# Autodesk Inventor assembly: 42146-11
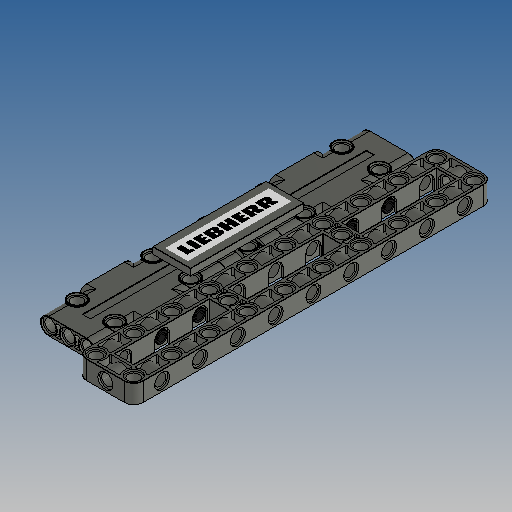
[picture p0: Inventor's stored thumbnail of the model, 512x512]
Saved by Autodesk Inventor 2025 (Build 290162010, 162A)
## iProperties
Created: 2024-11-18
Part Number: 42146-11
Material: Generisch
Document SubType Name: Assembly
Designer: hp.muther
Author: hp.muther
## Documents named in this file (7)
- D:\Inventor\Projekte\Muther\LEGO Technic\LEGO Technik - Raupenkran LR 13000 (42146)\42146-11.iam
- D:\Inventor\Projekte\Muther\LEGO Technic\LEGO Pieces\Verbindungselemente\39793-DkBluishGray.ipt
- D:\Inventor\Projekte\Muther\LEGO Technic\LEGO Pieces\Paneelen\71709-DkBluishGray.ipt
- D:\Inventor\Projekte\Muther\LEGO Technic\LEGO Pieces\Pin's\2780-Black.ipt
- D:\Inventor\Projekte\Muther\LEGO Technic\LEGO Pieces\Pin's\4274-Red.ipt
- D:\Inventor\Projekte\Muther\LEGO Technic\LEGO Pieces\Rahmen, T-Stücke\67491-DkBluishGray.ipt
- D:\Inventor\Projekte\Muther\LEGO Technic\LEGO Technik - Raupenkran LR 13000 (42146)\42146_69729_1.ipt
## Components (15 placed, 6 different names)
1. 39793-DkBluishGray:1 — Einfügen:1, Einfügen:2, Einfügen:3, Einfügen:4, Einfügen:5, Einfügen:6, Einfügen:7, Einfügen:12
2. 71709-DkBluishGray:1 — Einfügen:7, Einfügen:8, Einfügen:9, Passend:1, Passend:3
3. 2780-Black:1 — Einfügen:1, Passend:1
4. 2780-Black:2 — Einfügen:8
5. 2780-Black:3 — Einfügen:3
6. 2780-Black:4 — Einfügen:4, Passend:2
7. 2780-Black:5 — Einfügen:2
8. 2780-Black:6 — Einfügen:9
9. 4274-Red:1 — Einfügen:6, Passend:5
10. 4274-Red:2 — Einfügen:5, Einfügen:13
11. 71709-DkBluishGray:2 — Einfügen:12, Passend:2
12. 2780-Black:7 — Passend:4
13. 2780-Black:9
14. 67491-DkBluishGray:1 — Passend:3, Passend:4
15. 42146_69729_1:1 — Einfügen:13, Passend:5
## Relationships (18: Insert 13, Mate 5)
- Einfügen:1 [Insert]: 39793-DkBluishGray:1 ↔ 2780-Black:1
- Einfügen:2 [Insert]: 39793-DkBluishGray:1 ↔ 2780-Black:5
- Einfügen:3 [Insert]: 39793-DkBluishGray:1 ↔ 2780-Black:3
- Einfügen:4 [Insert]: 39793-DkBluishGray:1 ↔ 2780-Black:4
- Einfügen:5 [Insert]: 39793-DkBluishGray:1 ↔ 4274-Red:2
- Einfügen:6 [Insert]: 39793-DkBluishGray:1 ↔ 4274-Red:1
- Einfügen:7 [Insert]: 39793-DkBluishGray:1 ↔ 71709-DkBluishGray:1
- Einfügen:8 [Insert]: 71709-DkBluishGray:1 ↔ 2780-Black:2
- Einfügen:9 [Insert]: 71709-DkBluishGray:1 ↔ 2780-Black:6
- Passend:1 [Mate]: 71709-DkBluishGray:1 ↔ 2780-Black:1
- [Insert]: 71709-DkBluishGray:2 ↔ 2780-Black:7
- [Insert]: 71709-DkBluishGray:2 ↔ 2780-Black:9
- Einfügen:12 [Insert]: 39793-DkBluishGray:1 ↔ 71709-DkBluishGray:2
- Passend:2 [Mate]: 2780-Black:4 ↔ 71709-DkBluishGray:2
- Passend:3 [Mate]: 71709-DkBluishGray:1 ↔ 67491-DkBluishGray:1
- Passend:4 [Mate]: 2780-Black:7 ↔ 67491-DkBluishGray:1
- Einfügen:13 [Insert]: 4274-Red:2 ↔ 42146_69729_1:1
- Passend:5 [Mate]: 4274-Red:1 ↔ 42146_69729_1:1
## Named parameters: d10_d7 = 0 mm, d11_d8 = 0 mm
